# Autodesk Inventor assembly: TEST
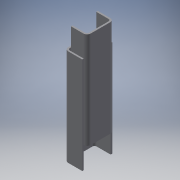
[picture p0: Inventor's stored thumbnail of the model, 180x180]
Saved by Autodesk Inventor 2017 (Build 210142000, 142)
## iProperties
Created: 2017-01-07
Part Number: TEST
Document SubType Name: Assembly
Designer: bramp
RuleStatus: InUse
Author: bramp
## Documents named in this file (3)
- D:\Gebruikers\bramp\Documents\Test\TEST.iam
- D:\Gebruikers\bramp\Documents\Test\Cprofiel.ipt
- D:\Gebruikers\bramp\Documents\Test\Poot.ipt
## Components (2 placed, 2 different names)
1. Cprofiel:1 — Mate:1, Mate:2, Mate:3
2. Poot:1 — Mate:1, Mate:2, Mate:3
## Relationships (3: Mate 3)
- Mate:1: Cprofiel:1 ↔ Poot:1
- Mate:2 (6 mm): Cprofiel:1 ↔ Poot:1
- Mate:3 (-140 mm): Cprofiel:1 ↔ Poot:1
